# Autodesk Inventor assembly: aktuator sa viljuskom
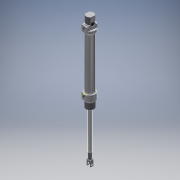
[picture p0: Inventor's stored thumbnail of the model, 180x180]
Saved by Autodesk Inventor 2019 (Build 230136000, 136)
## iProperties
Created: 2018-11-25
Part Number: aktuator sa viljuskom
Document SubType Name: Assembly
Designer: aleks
Author: aleks
## Documents named in this file (6)
- C:\Users\aleks\OneDrive\Desktop\novi klip\aktuator sa viljuskom.iam
- C:\Users\aleks\OneDrive\Desktop\novi klip\cilindar.ipt
- C:\Users\aleks\OneDrive\Desktop\novi klip\klipnjaca.ipt
- C:\Users\aleks\OneDrive\Desktop\novi klip\prednji deo assembly.iam
- C:\Users\aleks\OneDrive\Desktop\novi klip\zadnji deo assebly.iam
- C:\Users\aleks\OneDrive\Desktop\novi klip\prednja viljuska.ipt
## Components (5 placed, 5 different names)
1. klipnjaca:1 — Cylindrical:1, Insert:3
2. cilindar:1 — Cylindrical:1, Insert:1, Insert:2
3. prednji deo assembly:1 [sub-assembly] — Insert:1, Angle:1
4. zadnji deo assebly:1 [sub-assembly] — Insert:2, Angle:1
5. prednja viljuska:2 — Insert:3
## Relationships (5: Insert 3, CylindricalJoint 1, Angle 1)
- Cylindrical:1: klipnjaca:1 ↔ cilindar:1
- Insert:1: cilindar:1 ↔ prednji deo assembly:1
- Insert:2: cilindar:1 ↔ zadnji deo assebly:1
- Angle:1 (0 deg): prednji deo assembly:1 ↔ zadnji deo assebly:1
- Insert:3 (15 mm): klipnjaca:1 ↔ prednja viljuska:2
